# Autodesk Inventor assembly: nuc_w_bracket
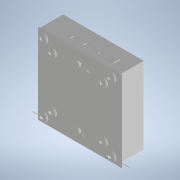
[picture p0: Inventor's stored thumbnail of the model, 180x180]
Saved by Autodesk Inventor 2020 (Build 240168000, 168)
## iProperties
Created: 2019-07-15
Part Number: nuc_w_bracket
Document SubType Name: Assembly
Designer: Senior Design
Author: Senior Design
## Documents named in this file (4)
- C:\Users\Senior Design\Documents\nuc_w_bracket.iam
- C:\Users\Senior Design\Documents\NUC_models\NUC_model.ipt
- C:\Users\Senior Design\Documents\NUC_models\nuc_mount_screw.ipt
- C:\Users\Senior Design\Documents\NUC_models\NUC_mount.ipt
## Components (4 placed, 3 different names)
1. NUC_model:1 — Flush:1, Flush:2, Flush:3, Mate:1, Mate:2, Mate:3, Mate:4
2. nuc_mount_screw:1 — Mate:1, Mate:4, Mate:6
3. nuc_mount_screw:2 — Mate:2, Mate:3, Mate:7, Mate:8
4. NUC_mount:1 — Mate:6, Mate:7, Mate:8
## Relationships (10: Mate 7, Flush 3)
- Flush:1: NUC_model:1
- Flush:2: NUC_model:1
- Flush:3: NUC_model:1
- Mate:1: NUC_model:1 ↔ nuc_mount_screw:1
- Mate:2: NUC_model:1 ↔ nuc_mount_screw:2
- Mate:3: NUC_model:1 ↔ nuc_mount_screw:2
- Mate:4: NUC_model:1 ↔ nuc_mount_screw:1
- Mate:6: nuc_mount_screw:1 ↔ NUC_mount:1
- Mate:7: nuc_mount_screw:2 ↔ NUC_mount:1
- Mate:8: nuc_mount_screw:2 ↔ NUC_mount:1
